# Autodesk Inventor assembly: SegaStraightAssembly
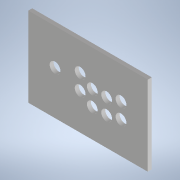
[picture p0: Inventor's stored thumbnail of the model, 180x180]
Saved by Autodesk Inventor 2022 (Build 260153000, 153)
## iProperties
Created: 2023-03-04
Part Number: SegaStraightAssembly
Document SubType Name: Assembly
Designer: Bunny
Author: Bunny
## Documents named in this file (2)
- C:\Users\Bunny\OneDrive - The University of Melbourne\project\controller\model\SegaStraightAssembly.iam
- C:\Users\Bunny\OneDrive - The University of Melbourne\project\controller\model\sega_straight.ipt
## Components (1 placed, 1 different names)
1. sega_straight:1
## Named parameters: BoxLength = 300 mm, BoxHeight = 80 mm, BoxWidth = 200 mm, SheetThickness = 6 mm, CornerOffset = 5 mm
